# Autodesk Inventor assembly: CAN
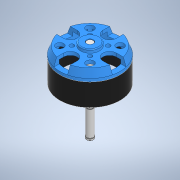
[picture p0: Inventor's stored thumbnail of the model, 180x180]
Saved by Autodesk Inventor 2022 (Build 260153000, 153)
## iProperties
Created: 2022-07-28
Part Number: CAN
Document SubType Name: Assembly
Designer: Nathan Cai
Author: Nathan Cai
## Documents named in this file (4)
- C:\Users\Nathan Cai\Documents\Inventor\Asorted Parts\Hobbyhh D3530 910KV\CAN.iam
- C:\Users\Nathan Cai\Documents\Inventor\Asorted Parts\Hobbyhh D3530 910KV\Top.ipt
- C:\Users\Nathan Cai\Documents\Inventor\Asorted Parts\Hobbyhh D3530 910KV\CAN.ipt
- C:\Users\Nathan Cai\Documents\Inventor\Asorted Parts\Hobbyhh D3530 910KV\SHAFT.ipt
## Components (3 placed, 3 different names)
1. Top:1 — Mate:1, Mate:2, Mate:3, Flush:1
2. CAN:1 — Mate:1, Mate:2
3. SHAFT:1 — Mate:3, Flush:1
## Relationships (4: Mate 3, Flush 1)
- Mate:1: Top:1 ↔ CAN:1
- Mate:2: Top:1 ↔ CAN:1
- Mate:3: Top:1 ↔ SHAFT:1
- Flush:1 (0.25 mm): Top:1 ↔ SHAFT:1
